# Autodesk Inventor assembly: kepala atas
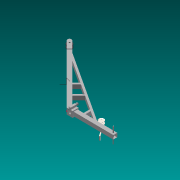
[picture p0: Inventor's stored thumbnail of the model, 180x180]
Saved by Autodesk Inventor 2014 SP2 (Build 180246200, 246)
## iProperties
Created: 2019-08-02
Part Number: kepala atas
Document SubType Name: Weldment
Designer: USER PC
Weld Material: Aluminum 6061, Welded
Author: USER PC
## Documents named in this file (6)
- C:\Users\USER PC\Desktop\United Tractors\New folder\kepala atas.iam
- C:\Users\USER PC\Desktop\United Tractors\New folder\pin kepala.ipt
- C:\Users\USER PC\Desktop\United Tractors\New folder\kepala baru.ipt
- C:\Users\USER PC\Desktop\United Tractors\New folder\Imported Components\Vints\Vints.ipt
- C:\Users\USER PC\Desktop\United Tractors\New folder\pulley.ipt
- C:\Users\USER PC\Desktop\United Tractors\New folder\pin pulley.ipt
## Components (5 placed, 5 different names)
1. pin kepala:1 — Mate:1
2. kepala baru:1 — Mate:1, Rigid:1, Rotational:1, Rotational:2
3. Vints:1 — Rigid:1
4. pulley:1 — Rotational:1
5. pin pulley:1 — Rotational:2
## Relationships (4: RevoluteJoint 2, Mate 1, WeldJoint 1)
- Mate:1: pin kepala:1 ↔ kepala baru:1
- Rigid:1 [WeldJoint]: kepala baru:1 ↔ Vints:1
- Rotational:1 [RevoluteJoint] (-5 mm): kepala baru:1 ↔ pulley:1
- Rotational:2 [RevoluteJoint] (20 mm): kepala baru:1 ↔ pin pulley:1
